# Autodesk Inventor assembly: prototype3
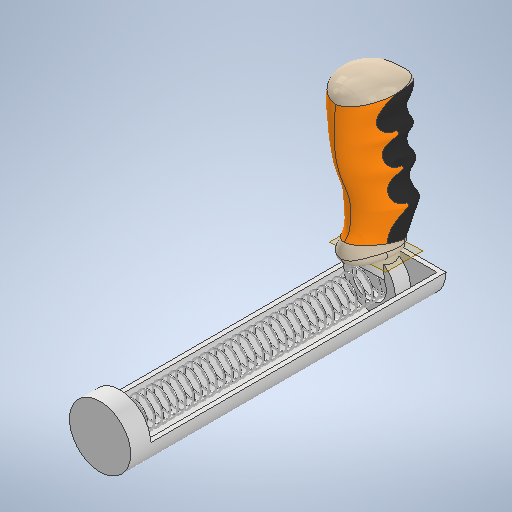
[picture p0: Inventor's stored thumbnail of the model, 512x512]
Saved by Autodesk Inventor 2025.1 (Build 291241020, 241B)
## iProperties
Created: 2024-11-22
Part Number: prototype3
Document SubType Name: Assembly
Designer: leon-
Author: leon-
## Documents named in this file (5)
- C:\Users\leon-\OneDrive\Dokumente\Education\Berkeley\Embedded_Systems\Project\MagDrop4\CAD_Model\3DPrint_Parts\Magazine_Test\prototype3.iam
- C:\Users\leon-\OneDrive\Dokumente\Education\Berkeley\Embedded_Systems\Project\MagDrop4\CAD_Model\3DPrint_Parts\Magazine_Test\prototype3_1.ipt
- C:\Users\leon-\OneDrive\Dokumente\Education\Berkeley\Embedded_Systems\Project\MagDrop4\CAD_Model\Purchase_Parts\Mechanical\Spring.ipt
- C:\Users\leon-\OneDrive\Dokumente\Education\Berkeley\Embedded_Systems\Project\MagDrop4\CAD_Model\3DPrint_Parts\Magazine_Test\prototype3_2.ipt
- C:\Users\leon-\OneDrive\Dokumente\Education\Berkeley\Embedded_Systems\Project\MagDrop4\CAD_Model\3DPrint_Parts\Magazine_Test\GRIP  5.ipt
## Components (4 placed, 4 different names)
1. prototype3_1:1 — Mate:1, Mate:2, Mate:3, Angle:1
2. Spring:1 — Mate:1, Mate:2, Mate:4
3. prototype3_2:1 — Mate:3, Mate:4, Mate:5, Mate:6
4. GRIP  5:1 — Mate:5, Mate:6, Angle:1
## Relationships (7: Mate 6, Angle 1)
- Mate:1: prototype3_1:1 ↔ Spring:1
- Mate:2: prototype3_1:1 ↔ Spring:1
- Mate:3: prototype3_1:1 ↔ prototype3_2:1
- Mate:4: Spring:1 ↔ prototype3_2:1
- Mate:5: prototype3_2:1 ↔ GRIP  5:1
- Mate:6: prototype3_2:1 ↔ GRIP  5:1
- Angle:1 (180 deg): prototype3_1:1 ↔ GRIP  5:1
